# Autodesk Inventor assembly: s-assy-frame-connector
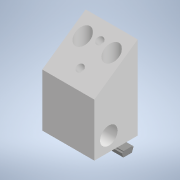
[picture p0: Inventor's stored thumbnail of the model, 180x180]
Saved by Autodesk Inventor 2022 (Build 260153000, 153)
## iProperties
Created: 2021-09-21
Part Number: s-assy-frame-connector
Document SubType Name: Assembly
Designer: yuto6
Author: yuto6
## Documents named in this file (4)
- C:\Users\yuto6\Box\Public_Share\キャチロボバトルコンテスト2021\CAD\catchrobo_hardware\assy-shooter\s-assy-frame-connector.iam
- C:\Users\yuto6\Box\Public_Share\キャチロボバトルコンテスト2021\CAD\catchrobo_hardware\assy-shooter\s_base1_2.ipt
- C:\Users\yuto6\Box\Public_Share\キャチロボバトルコンテスト2021\CAD\catchrobo_hardware\assy-shooter\HNTP5-5_app.ipt
- C:\Users\yuto6\Box\Public_Share\キャチロボバトルコンテスト2021\CAD\catchrobo_hardware\assy-shooter\CB5-35.ipt
## Components (5 placed, 3 different names)
1. s_base1_2:1 — メイト:1, メイト:2, 角度:1, 角度:2, フラッシュ:1, フラッシュ:2, メイト:3, メイト:4, メイト:5, メイト:6
2. HNTP5-5_app:1 — メイト:2, フラッシュ:2, 角度:2
3. HNTP5-5_app:2 — メイト:1, 角度:1, フラッシュ:1
4. CB5-35:1 — メイト:3, メイト:6
5. CB5-35:2 — メイト:4, メイト:5
## Relationships (10: Mate 6, Angle 2, Flush 2)
- メイト:1 [Mate]: s_base1_2:1 ↔ HNTP5-5_app:2
- メイト:2 [Mate]: s_base1_2:1 ↔ HNTP5-5_app:1
- 角度:1 [Angle] (0 deg): s_base1_2:1 ↔ HNTP5-5_app:2
- 角度:2 [Angle] (0 deg): s_base1_2:1 ↔ HNTP5-5_app:1
- フラッシュ:1 [Flush] (5.2 mm): s_base1_2:1 ↔ HNTP5-5_app:2
- フラッシュ:2 [Flush] (5.2 mm): s_base1_2:1 ↔ HNTP5-5_app:1
- メイト:3 [Mate]: s_base1_2:1 ↔ CB5-35:1
- メイト:4 [Mate]: s_base1_2:1 ↔ CB5-35:2
- メイト:5 [Mate]: s_base1_2:1 ↔ CB5-35:2
- メイト:6 [Mate]: s_base1_2:1 ↔ CB5-35:1
